# Autodesk Inventor assembly: ASY дренаж угольные
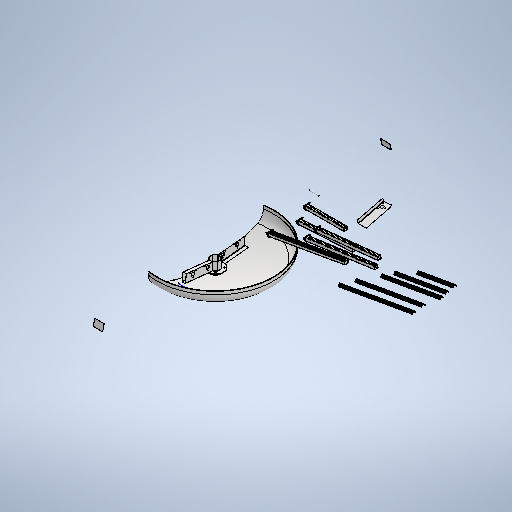
[picture p0: Inventor's stored thumbnail of the model, 512x512]
Saved by Autodesk Inventor 2025 (Build 290162010, 162A)
## iProperties
Created: 2024-12-09
Part Number: ASY дренаж угольные
Document SubType Name: Assembly
Designer: user
Author: user
## Documents named in this file (24)
- C:\Users\admin\YandexDisk-badmisterfox\home pc\Inventor\filter  distribution system\ASY BOTTOM filter distribution system.iam
- C:\Users\admin\YandexDisk-badmisterfox\home pc\Inventor\filter  distribution system\drain flange.ipt
- C:\Users\admin\YandexDisk-badmisterfox\home pc\Inventor\filter  distribution system\Фильтр напорный угольный 30 куб час.ipt
- C:\Users\admin\YandexDisk-badmisterfox\home pc\Inventor\filter  distribution system\MNT-CDF-401 roof 975.ipt
- C:\Users\admin\YandexDisk-badmisterfox\home pc\Inventor\filter  distribution system\MNT-CDF-501 box.ipt
- C:\Users\admin\YandexDisk-badmisterfox\home pc\Inventor\filter  distribution system\MNT-CDF-502 tube.ipt
- C:\Users\admin\YandexDisk-badmisterfox\home pc\Inventor\filter  distribution system\MNT-CDF-503  main tube 1.ipt
- C:\Users\admin\YandexDisk-badmisterfox\home pc\Inventor\Manturovo\Content Center Files\en-US\DIN 933\DIN 933 - M8  x 20.ipt
- C:\Users\admin\YandexDisk-badmisterfox\home pc\Inventor\filter  distribution system\MNT-CDF-504 small tube flange.ipt
- C:\Users\admin\YandexDisk-badmisterfox\home pc\Inventor\filter  distribution system\MNT-CDF-315 beam 5.ipt
- C:\Users\admin\YandexDisk-badmisterfox\home pc\Inventor\filter  distribution system\MNT-CDF-312 beam 2.ipt
- C:\Users\admin\YandexDisk-badmisterfox\home pc\Inventor\filter  distribution system\MNT-CDF-313 beam 3.ipt
- C:\Users\admin\YandexDisk-badmisterfox\home pc\Inventor\filter  distribution system\MNT-CDF-314 beam 4.ipt
- C:\Users\admin\YandexDisk-badmisterfox\home pc\Inventor\filter  distribution system\MNT-CDF-601 CAP.ipt
- C:\Users\admin\YandexDisk-badmisterfox\home pc\Inventor\filter  distribution system\MNT-CDF-602 CAP.ipt
- C:\Users\admin\YandexDisk-badmisterfox\home pc\Inventor\filter  distribution system\MNT-CDF-603 CAP.ipt
- C:\Users\admin\YandexDisk-badmisterfox\home pc\Inventor\filter  distribution system\ASY Луч 1.iam
- C:\Users\admin\YandexDisk-badmisterfox\home pc\Inventor\filter  distribution system\MNT-CDF-402 roof 875.ipt
- C:\Users\admin\YandexDisk-badmisterfox\home pc\Inventor\filter  distribution system\MNT-CDF-403 roof 775.ipt
- C:\Users\admin\YandexDisk-badmisterfox\home pc\Inventor\filter  distribution system\MNT-CDF-404 roof 675.ipt
- C:\Users\admin\YandexDisk-badmisterfox\home pc\Inventor\filter  distribution system\MNT-CDF-405 roof 475.ipt
- C:\Users\admin\YandexDisk-badmisterfox\home pc\Inventor\filter  distribution system\000 DS-B dimentions.ipt
- C:\Users\admin\YandexDisk-badmisterfox\home pc\Inventor\filter  distribution system\000 DS-B outer tube.ipt
- C:\Users\admin\YandexDisk-badmisterfox\home pc\Inventor\filter  distribution system\110 DS-B drain sustem flange.ipt
## Components (35 placed, 23 different names)
1. 000 DS-B dimentions:1
2. Фильтр напорный угольный 30 куб час:1 — Mate:4, Flush:3, Flush:4, Rigid:36
3. MNT-CDF-501 box:1 — Mate:5, Flush:5, Mate:6, Rigid:40
4. drain flange:2 — Rigid:37
5. MNT-CDF-502 tube:4
6. MNT-CDF-502 tube:3
7. MNT-CDF-502 tube:2
8. MNT-CDF-503  main tube 1:1 — Rigid:39, Mate:7
9. MNT-CDF-503  main tube 1:2 — Mate:5, Rigid:38
10. MNT-CDF-501 box:2 — Mate:7, Mate:8, Mate:9
11. DIN 933 - replaced by DIN EN 24017 M8  x 20:1
12. MNT-CDF-502 tube:5
13. MNT-CDF-315 beam 5:1 — Rigid:21
14. Part1:5 — Rigid:21
15. DIN 933 - replaced by DIN EN 24017 M8  x 20:2
16. DIN 933 - replaced by DIN EN 24017 M8  x 20:3
17. MNT-CDF-312 beam 2:1 — Rigid:26
18. Part1:6 — Rigid:26
19. Part1:7 — Rigid:27
20. Part1:8 — Rigid:28
21. MNT-CDF-313 beam 3:1 — Rigid:27
22. MNT-CDF-314 beam 4:1 — Rigid:28
23. MNT-CDF-601 CAP:1
24. MNT-CDF-602 CAP:1
25. MNT-CDF-602 CAP:2
26. MNT-CDF-603 CAP:1 — Rigid:40
27. MNT-CDF-603 CAP:2
28. ASY Луч 1:1 [sub-assembly]
29. MNT-CDF-401 roof 975:1
30. MNT-CDF-402 roof 875:1
31. MNT-CDF-403 roof 775:1
32. MNT-CDF-404 roof 675:1
33. MNT-CDF-405 roof 475:1
34. 000 DS-B outer tube:1 — Rigid:36, Rigid:37
35. drain sustem flange:1 — Mate:6, Rigid:38, Rigid:39, Mate:8
## Relationships (21: WeldJoint 9, Mate 6, Flush 3, RevoluteJoint 3)
- Mate:4: Фильтр напорный угольный 30 куб час:1
- Flush:3: Фильтр напорный угольный 30 куб час:1
- Flush:4: Фильтр напорный угольный 30 куб час:1
- Rigid:21 [WeldJoint]: MNT-CDF-315 beam 5:1 ↔ Part1:5
- Rigid:26 [WeldJoint]: MNT-CDF-312 beam 2:1 ↔ Part1:6
- Rigid:27 [WeldJoint]: Part1:7 ↔ MNT-CDF-313 beam 3:1
- Rigid:28 [WeldJoint]: Part1:8 ↔ MNT-CDF-314 beam 4:1
- [RevoluteJoint]: DIN 933 - replaced by DIN EN 24017 M8  x 20:2 ↔ ASY Луч 1:1
- [RevoluteJoint]: DIN 933 - replaced by DIN EN 24017 M8  x 20:3 ↔ ASY Луч 1:1
- [RevoluteJoint]: DIN 933 - replaced by DIN EN 24017 M8  x 20:1 ↔ ASY Луч 1:1
- Rigid:36 [WeldJoint]: Фильтр напорный угольный 30 куб час:1 ↔ 000 DS-B outer tube:1
- Rigid:37 [WeldJoint]: drain flange:2 ↔ 000 DS-B outer tube:1
- Mate:5: MNT-CDF-501 box:1 ↔ MNT-CDF-503  main tube 1:2
- Flush:5: MNT-CDF-501 box:1
- Mate:6: MNT-CDF-501 box:1 ↔ drain sustem flange:1
- Rigid:38 [WeldJoint]: MNT-CDF-503  main tube 1:2 ↔ drain sustem flange:1
- Rigid:39 [WeldJoint]: MNT-CDF-503  main tube 1:1 ↔ drain sustem flange:1
- Mate:7: MNT-CDF-503  main tube 1:1 ↔ MNT-CDF-501 box:2
- Mate:8: MNT-CDF-501 box:2 ↔ drain sustem flange:1
- Mate:9: MNT-CDF-501 box:2
- Rigid:40 [WeldJoint]: MNT-CDF-501 box:1 ↔ MNT-CDF-603 CAP:1
